# Autodesk Inventor assembly: Assembly1
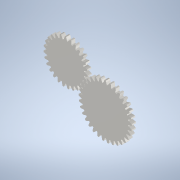
[picture p0: Inventor's stored thumbnail of the model, 180x180]
Saved by Autodesk Inventor 2020.1 (Build 241239000, 239)
## iProperties
Created: 2020-02-22
Part Number: Assembly1
Document SubType Name: Assembly
Designer: Ali
Author: Ali
## Documents named in this file (3)
- F:\Inventor_Projects\AlorsBot_CAD\inventor\assemblies\Assembly1.iam
- F:\Inventor_Projects\AlorsBot_CAD\inventor\assemblies\Assembly1\Design Accelerator\Spur Gears4.iam
- F:\Inventor_Projects\AlorsBot_CAD\inventor\excel\wheelParameters.xlsx
## Components (1 placed, 1 different names)
1. Spur Gears:1 [sub-assembly]
## Named parameters: Wheel_Related_W_ = 0, W_innerDiameter = 70 mm, W_innerDepth = 4 mm, W_wallThickness = 2 mm, W_holesClearance = 0.3 mm, W_outerGearHoleDiameter = 5.3 mm, W_innerGearHoleDiameter = 10.1 mm, W_filletRadius = 0.25 mm, W_numberOfSlits = 4, W_extrutsionTaperAngle = 2 deg, Reserved_10 = 0 mm, Inner_Gear_Related_IG_ = 0, IG_ratioToOuterGear = 0.5, IG_gearDiameter = 20 mm, IG_gearThickness = 2 mm, IG_shaftDiameter = 7.5 mm, IG_shaftLength = 17 mm, IG_skirtOffset = 10 mm, IG_skirtThickness = 2 mm, IG_extentionLength = 19.5 mm, IG_extentionThickness = 3 mm, IG_slitDistanceFromCenterHole = 7 mm, IG_slitClearance = 0.2 mm, IG_slitWidth = 4 mm, IG_slitlength = 8 mm, IG_dAxleCircleDiameter = 2 mm, IG_dAxleShort = 1.5 mm, IG_dAxleDepth = 5 mm, Outer_Gear_Related_OG_ = 0, OG_distanceFromCenter = 22.5 mm, OG_gearDiameter = 25 mm, OG_gearThickness = 2 mm, OG_shaftDiameter = 5 mm, OG_shaftLength = 9 mm, OG_skirtOffset = 5 mm, OG_skirtThickness = 1 mm, OG_numberOfGears = 5, OG_protrudeDistance = 3 mm, Reserved_12 = 0 mm, Leg_Extensions_Related_LE_ = 0, LE_baseDiameter = 5 mm, LE_thickness = 2.5 mm, LE_maxLength = 23.67256 mm, LE_offsetAboveOuterGear = 0 mm, Reserved_13 = 0 mm, Reserved_14 = 0 mm, Reserved_15 = 0 mm, Reserved_16 = 0 mm, Reserved_17 = 0 mm, Reserved_18 = 0 mm, Bearing_Related_BR_ = 0, BR_bearingThickness = 1 mm, Reserved_19 = 0 mm, Reserved_20 = 0 mm, Reserved_21 = 0 mm, Reserved_22 = 0 mm, Block_Related_BL_ = 0, BL_width = 3.8 mm, BL_length = 7.8 mm, BL_depth = 10 mm, Reserved_23 = 0 mm, Reserved_24 = 0 mm, Reserved_25 = 0 mm, Reserved_26 = 0 mm, Reserved_27 = 0 mm, IG_gearRatio = 1.25
